# Autodesk Inventor assembly: Zespół1
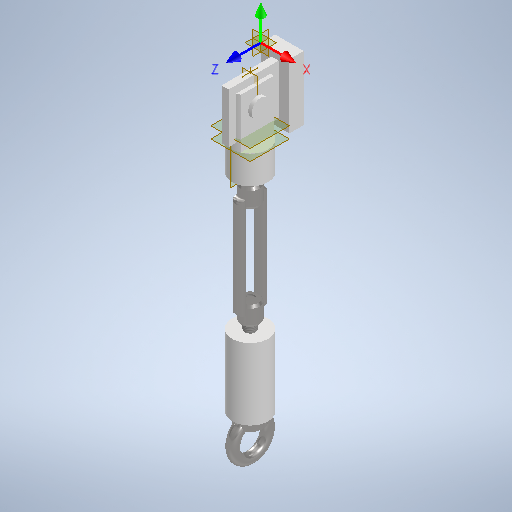
[picture p0: Inventor's stored thumbnail of the model, 512x512]
Saved by Autodesk Inventor 2025.2 (Build 292293000, 293)
## iProperties
Created: 2025-04-28
Part Number: Zespół1
Document SubType Name: Assembly
Designer: marci
Author: marci
## Documents named in this file (9)
- D:\Podstawy-Konstrukcji-Maszyn\Projekt2_temat4.1\Zespół1.iam
- D:\Podstawy-Konstrukcji-Maszyn\Projekt2_temat4.1\przegub.ipt
- D:\Podstawy-Konstrukcji-Maszyn\Projekt2_temat4.1\rama_1.ipt
- D:\Podstawy-Konstrukcji-Maszyn\Projekt2_temat4.1\rama_2.ipt
- D:\Podstawy-Konstrukcji-Maszyn\Projekt2_temat4.1\sworzeń.ipt
- D:\Podstawy-Konstrukcji-Maszyn\Projekt2_temat4.1\content_center\pl-PL\DIN 1480\DIN 1480 - _SP - M16.ipt
- D:\Podstawy-Konstrukcji-Maszyn\Projekt2_temat4.1\content_center\pl-PL\DIN 976-1 A\DIN 976-1 - M16 x 60 - A.ipt
- D:\Podstawy-Konstrukcji-Maszyn\Projekt2_temat4.1\mocowanie_pod_hak.ipt
- D:\Podstawy-Konstrukcji-Maszyn\Projekt2_temat4.1\content_center\pl-PL\CNS 4491\CNS 4491 - M16 x 1,5 x 27 - 1,2.ipt
## Components (9 placed, 8 different names)
1. przegub:1 — Obrotowe:1, Obrotowe:2, Walcowe:5
2. rama_1:1 — Zestawiające:1, Równoległe:1, Równoległe:2, Obrotowe:1
3. rama_2:1 — Zestawiające:4, Zestawiające:9, Równoległe:3, Zestawiające:1, Równoległe:1, Równoległe:2
4. sworzeń:1 — Obrotowe:2
5. DIN 1480 SP - M16:1 — Walcowe:1, Walcowe:2
6. DIN 976-1 A M16 x 60:1 — Walcowe:5, Walcowe:1
7. DIN 976-1 A M16 x 60:2 — Walcowe:2, Walcowe:3
8. mocowanie_pod_hak:1 — Walcowe:3, Walcowe:4
9. CNS 4491 M16 x 27:1 — Walcowe:4
## Relationships (19: Mate 9, CylindricalJoint 5, Flush 3, RevoluteJoint 2)
- Zestawiające:2 [Mate]
- Zestawiające:6 [Mate]
- Zestawiające:5 [Mate]
- Zestawiające:8 [Mate]
- Zestawiające:7 [Mate]
- Zestawiające:3 [Mate]
- Zestawiające:4 [Mate]: rama_2:1
- Zestawiające:9 [Mate]: rama_2:1
- Równoległe:3 [Flush]: rama_2:1
- Zestawiające:1 [Mate]: rama_1:1 ↔ rama_2:1
- Równoległe:1 [Flush] (9.192 mm): rama_1:1 ↔ rama_2:1
- Równoległe:2 [Flush] (15 mm): rama_1:1 ↔ rama_2:1
- Obrotowe:1 [RevoluteJoint]: przegub:1 ↔ rama_1:1
- Obrotowe:2 [RevoluteJoint] (-5 mm): przegub:1 ↔ sworzeń:1
- Walcowe:5 [CylindricalJoint]: przegub:1 ↔ DIN 976-1 A M16 x 60:1
- Walcowe:1 [CylindricalJoint]: DIN 1480 SP - M16:1 ↔ DIN 976-1 A M16 x 60:1
- Walcowe:2 [CylindricalJoint]: DIN 1480 SP - M16:1 ↔ DIN 976-1 A M16 x 60:2
- Walcowe:3 [CylindricalJoint]: DIN 976-1 A M16 x 60:2 ↔ mocowanie_pod_hak:1
- Walcowe:4 [CylindricalJoint]: mocowanie_pod_hak:1 ↔ CNS 4491 M16 x 27:1
